# Autodesk Inventor assembly: H-Connector_2020-asm
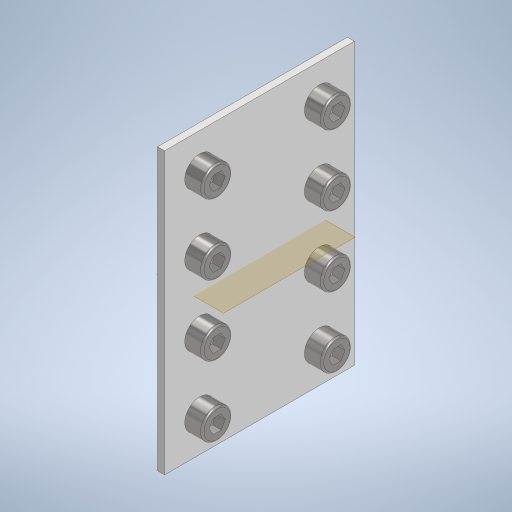
[picture p0: Inventor's stored thumbnail of the model, 512x512]
Saved by Autodesk Inventor 2024 (Build 280153000, 153)
## iProperties
Created: 2025-12-25
Part Number: H-Connector_2020-asm
Document SubType Name: Assembly
Designer: schar
Author: schar
## Documents named in this file (4)
- C:\Users\schar\Desktop\projectBlueprint\AMSTS\hardware\H-Connector_2020-asm.iam
- C:\Users\schar\Desktop\projectBlueprint\AMSTS\hardware\H-Connector_2020.ipt
- C:\Users\schar\Desktop\projectBlueprint\AMSTS\hardware\tnut_m5_2020.ipt
- C:\Users\schar\Documents\Inventor\Content Center Files\R2024\en-US\ISO 4762(1)\DIN EN ISO 4762 - M5 x 8.ipt
## Components (17 placed, 3 different names)
1. H-Connector_2020:1 — Rigid:1, Rigid:2, Rigid:3, Rigid:4, Rigid:5, Rigid:6, Rigid:7, Rigid:8, Mate:1, Mate:2, Mate:3, Mate:4, Mate:5, Mate:6, Mate:7, Mate:8, Mate:9, Mate:18, Mate:19, Mate:20, Mate:21
2. tnut_m5_2020:3 — Rigid:1, Mate:14
3. tnut_m5_2020:4 — Rigid:4, Mate:17
4. tnut_m5_2020:7 — Rigid:2, Mate:15
5. tnut_m5_2020:8 — Rigid:3, Mate:16
6. tnut_m5_2020:9 — Rigid:5, Mate:10
7. tnut_m5_2020:10 — Rigid:6, Mate:12
8. tnut_m5_2020:11 — Rigid:7, Mate:11
9. tnut_m5_2020:12 — Rigid:8, Mate:13
10. DIN EN ISO 4762 M5 x 8:1 — Mate:6, Mate:17
11. DIN EN ISO 4762 M5 x 8:2 — Mate:7, Mate:15
12. DIN EN ISO 4762 M5 x 8:3 — Mate:8, Mate:13
13. DIN EN ISO 4762 M5 x 8:4 — Mate:9, Mate:11
14. DIN EN ISO 4762 M5 x 8:5 — Mate:2, Mate:16
15. DIN EN ISO 4762 M5 x 8:6 — Mate:3, Mate:14
16. DIN EN ISO 4762 M5 x 8:7 — Mate:4, Mate:12
17. DIN EN ISO 4762 M5 x 8:8 — Mate:5, Mate:10
## Relationships (34: Mate 25, WeldJoint 8, Symmetry 1)
- Rigid:1 [WeldJoint] (0.159 mm): H-Connector_2020:1 ↔ tnut_m5_2020:3
- Rigid:2 [WeldJoint] (0.159 mm): H-Connector_2020:1 ↔ tnut_m5_2020:7
- Rigid:3 [WeldJoint] (0.159 mm): H-Connector_2020:1 ↔ tnut_m5_2020:8
- Rigid:4 [WeldJoint] (0.159 mm): H-Connector_2020:1 ↔ tnut_m5_2020:4
- Rigid:5 [WeldJoint] (0.159 mm): H-Connector_2020:1 ↔ tnut_m5_2020:9
- Rigid:6 [WeldJoint] (0.159 mm): H-Connector_2020:1 ↔ tnut_m5_2020:10
- Rigid:7 [WeldJoint] (0.159 mm): H-Connector_2020:1 ↔ tnut_m5_2020:11
- Rigid:8 [WeldJoint] (0.159 mm): H-Connector_2020:1 ↔ tnut_m5_2020:12
- Mate:1: H-Connector_2020:1
- Mate:2: H-Connector_2020:1 ↔ DIN EN ISO 4762 M5 x 8:5
- Mate:3: H-Connector_2020:1 ↔ DIN EN ISO 4762 M5 x 8:6
- Mate:4: H-Connector_2020:1 ↔ DIN EN ISO 4762 M5 x 8:7
- Mate:5: H-Connector_2020:1 ↔ DIN EN ISO 4762 M5 x 8:8
- Mate:6: H-Connector_2020:1 ↔ DIN EN ISO 4762 M5 x 8:1
- Mate:7: H-Connector_2020:1 ↔ DIN EN ISO 4762 M5 x 8:2
- Mate:8: H-Connector_2020:1 ↔ DIN EN ISO 4762 M5 x 8:3
- Mate:9: H-Connector_2020:1 ↔ DIN EN ISO 4762 M5 x 8:4
- Mate:10: tnut_m5_2020:9 ↔ DIN EN ISO 4762 M5 x 8:8
- Mate:11: tnut_m5_2020:11 ↔ DIN EN ISO 4762 M5 x 8:4
- Mate:12: tnut_m5_2020:10 ↔ DIN EN ISO 4762 M5 x 8:7
- Mate:13: tnut_m5_2020:12 ↔ DIN EN ISO 4762 M5 x 8:3
- Mate:14: tnut_m5_2020:3 ↔ DIN EN ISO 4762 M5 x 8:6
- Mate:15: tnut_m5_2020:7 ↔ DIN EN ISO 4762 M5 x 8:2
- Mate:16: tnut_m5_2020:8 ↔ DIN EN ISO 4762 M5 x 8:5
- Mate:17: tnut_m5_2020:4 ↔ DIN EN ISO 4762 M5 x 8:1
- Mate:18: H-Connector_2020:1
- Mate:19: H-Connector_2020:1
- Mate:20: H-Connector_2020:1
- Mate:21: H-Connector_2020:1
- Mate:22
- Mate:23
- Mate:24
- Mate:25
- Symmetry:1
